# Autodesk Inventor assembly: 8163946 CMMT-ST-C8-1C-MP-S0---(high)
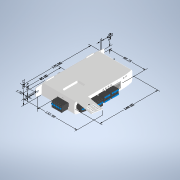
[picture p0: Inventor's stored thumbnail of the model, 180x180]
Saved by Autodesk Inventor 2021 (Build 250183000, 183)
## iProperties
Category: PARTsolutions
Company: FESTO
Created: 2026-04-23
Part Number: 8163946 CMMT-ST-C8-1C-MP-S0---(high)
Catalog Web Link: www.3dfindit.com
Description: CMMT-ST-servo drive
Vendor: FESTO
Document SubType Name: Assembly
Designer: psAdmin
Manufacturer: FESTO
Mass: 350 g
Surface Area: 725.969 cm^2
Volume: 348.658 cm^3
Density: 1.00385 g/cm^3
Title: 8163946 CMMT-ST-C8-1C-MP-S0
Author: Cadenas PARTsolutions
Comments: servo drive
PSOL_IDENT_0: {ATYP=ASSISTANT},{DATA=script=$CADENAS_DATA/23d-libs/festo/webfesto.vbb&M_FAMILY=CMMT&M_GROUP=01&M_P
PSOL_IDENT_1: ARTNO=8163946&IDCODE1=CMMT-ST-C8-1C-MP-S0&IDCODE2=&customer_number_cns=&MATES=1&LOD=HI&LOCKERP=0&SIN
PSOL_IDENT_2: GLEPART=1}
NB: 8163946 CMMT-ST-C8-1C-MP-S0---(high)
NN: CMMT-ST
NT: servo drive
NBSYN: $TNR. $TYP.---($LODLEVEL.)
LINA: 8163946 CMMT-ST-C8-1C-MP-S0
CATALOG: Festo
TNR: 8163946
TYP: CMMT-ST-C8-1C-MP-S0
LODLEVEL: High
CNSMASSEXACT: 0.35
GTIN: 4052568631956
SUPPLIER: FESTO
ARTICLENO: 8163946 CMMT-ST-C8-1C-MP-S0---(high)
BOMINFO: 8163946 CMMT-ST-C8-1C-MP-S0
CREATOR: CADENAS GmbH
## Documents named in this file (9)
- e:\temp\worker_COMMON_66\temp\tmp_7696_12_FVe9l\format_0\8163946 CMMT-ST-C8-1C-MP-S0---(high).iam
- e:\temp\worker_COMMON_66\temp\tmp_7696_12_FVe9l\format_0\8163946 CMMT-ST-C8-1C-MP-S0---(highh).ipt
- e:\temp\worker_COMMON_66\temp\tmp_7696_12_FVe9l\format_0\1360395 VAME-P11-MK.ipt
- e:\temp\worker_COMMON_66\temp\tmp_7696_12_FVe9l\format_0\DIN-912 - M4x5(F).ipt
- e:\temp\worker_COMMON_66\temp\tmp_7696_12_FVe9l\format_0\8079510 10GD-2RR3,5-CLP-CBL.ipt
- e:\temp\worker_COMMON_66\temp\tmp_7696_12_FVe9l\format_0\8079513 8GD-2RR3,5-CLP-CBL.ipt
- e:\temp\worker_COMMON_66\temp\tmp_7696_12_FVe9l\format_0\8079509 6GD-1RR5,08-CLP-CBL.ipt
- e:\temp\worker_COMMON_66\temp\tmp_7696_12_FVe9l\format_0\8079508 3GD-1RR3_5-CLP-CBL---(2).ipt
- e:\temp\worker_COMMON_66\temp\tmp_7696_12_FVe9l\format_0\8169608 5GD-1RR5,08-CLP-CBL.ipt
## Components (8 placed, 8 different names)
1. 8163946 CMMT-ST-C8-1C-MP-S0---(highh):1 — IP1_XY@1 <-> N_XY@2, IP1_Z@1 <-> N_Z@2, IP1_YZ@1 <-> N_YZ@2, P1_XY@1 <-> CP1_XY@4, P1_Z@1 <-> CP1_Z@4, P1_YZ@1 <-> CP1_YZ@4, P2_XY@1 <-> CP1_XY@5, P2_Z@1 <-> CP1_Z@5, P2_YZ@1 <-> CP1_YZ@5, P3_XY@1 <-> CP1_XY@6, P3_Z@1 <-> CP1_Z@6, P3_YZ@1 <-> CP1_YZ@6, P4_XY@1 <-> CP1_XY@7, P4_Z@1 <-> CP1_Z@7, P4_YZ@1 <-> CP1_YZ@7, P5_XY@1 <-> CP1_XY@8, P5_Z@1 <-> CP1_Z@8, P5_YZ@1 <-> CP1_YZ@8
2. 1360395 VAME-P11-MK:1 — IP1_XY@1 <-> N_XY@2, IP1_Z@1 <-> N_Z@2, IP1_YZ@1 <-> N_YZ@2, B_XY@2 <-> ANBAU_XY@3, B_Z@2 <-> ANBAU_Z@3, B_YZ@2 <-> ANBAU_YZ@3
3. DIN-912 - M4x5(F):1 — B_XY@2 <-> ANBAU_XY@3, B_Z@2 <-> ANBAU_Z@3, B_YZ@2 <-> ANBAU_YZ@3
4. 8079510 10GD-2RR3,5-CLP-CBL:1 — P1_XY@1 <-> CP1_XY@4, P1_Z@1 <-> CP1_Z@4, P1_YZ@1 <-> CP1_YZ@4
5. 8079513 8GD-2RR3,5-CLP-CBL:1 — P2_XY@1 <-> CP1_XY@5, P2_Z@1 <-> CP1_Z@5, P2_YZ@1 <-> CP1_YZ@5
6. 8079509 6GD-1RR5,08-CLP-CBL:1 — P3_XY@1 <-> CP1_XY@6, P3_Z@1 <-> CP1_Z@6, P3_YZ@1 <-> CP1_YZ@6
7. 8079508 3GD-1RR3_5-CLP-CBL---(2):1 — P4_XY@1 <-> CP1_XY@7, P4_Z@1 <-> CP1_Z@7, P4_YZ@1 <-> CP1_YZ@7
8. 8169608 5GD-1RR5,08-CLP-CBL:1 — P5_XY@1 <-> CP1_XY@8, P5_Z@1 <-> CP1_Z@8, P5_YZ@1 <-> CP1_YZ@8
## Relationships (21: Mate 13, Angle 7, Flush 1)
- IP1_XY@1 <-> N_XY@2 [Mate] (1.35 mm): 8163946 CMMT-ST-C8-1C-MP-S0---(highh):1 ↔ 1360395 VAME-P11-MK:1
- IP1_Z@1 <-> N_Z@2 [Mate]: 8163946 CMMT-ST-C8-1C-MP-S0---(highh):1 ↔ 1360395 VAME-P11-MK:1
- IP1_YZ@1 <-> N_YZ@2 [Angle] (0 deg): 8163946 CMMT-ST-C8-1C-MP-S0---(highh):1 ↔ 1360395 VAME-P11-MK:1
- B_XY@2 <-> ANBAU_XY@3 [Flush]: 1360395 VAME-P11-MK:1 ↔ DIN-912 - M4x5(F):1
- B_Z@2 <-> ANBAU_Z@3 [Mate]: 1360395 VAME-P11-MK:1 ↔ DIN-912 - M4x5(F):1
- B_YZ@2 <-> ANBAU_YZ@3 [Angle] (0 deg): 1360395 VAME-P11-MK:1 ↔ DIN-912 - M4x5(F):1
- P1_XY@1 <-> CP1_XY@4 [Mate]: 8163946 CMMT-ST-C8-1C-MP-S0---(highh):1 ↔ 8079510 10GD-2RR3,5-CLP-CBL:1
- P1_Z@1 <-> CP1_Z@4 [Mate]: 8163946 CMMT-ST-C8-1C-MP-S0---(highh):1 ↔ 8079510 10GD-2RR3,5-CLP-CBL:1
- P1_YZ@1 <-> CP1_YZ@4 [Angle] (0 deg): 8163946 CMMT-ST-C8-1C-MP-S0---(highh):1 ↔ 8079510 10GD-2RR3,5-CLP-CBL:1
- P2_XY@1 <-> CP1_XY@5 [Mate]: 8163946 CMMT-ST-C8-1C-MP-S0---(highh):1 ↔ 8079513 8GD-2RR3,5-CLP-CBL:1
- P2_Z@1 <-> CP1_Z@5 [Mate]: 8163946 CMMT-ST-C8-1C-MP-S0---(highh):1 ↔ 8079513 8GD-2RR3,5-CLP-CBL:1
- P2_YZ@1 <-> CP1_YZ@5 [Angle] (0 deg): 8163946 CMMT-ST-C8-1C-MP-S0---(highh):1 ↔ 8079513 8GD-2RR3,5-CLP-CBL:1
- P3_XY@1 <-> CP1_XY@6 [Mate]: 8163946 CMMT-ST-C8-1C-MP-S0---(highh):1 ↔ 8079509 6GD-1RR5,08-CLP-CBL:1
- P3_Z@1 <-> CP1_Z@6 [Mate]: 8163946 CMMT-ST-C8-1C-MP-S0---(highh):1 ↔ 8079509 6GD-1RR5,08-CLP-CBL:1
- P3_YZ@1 <-> CP1_YZ@6 [Angle] (0 deg): 8163946 CMMT-ST-C8-1C-MP-S0---(highh):1 ↔ 8079509 6GD-1RR5,08-CLP-CBL:1
- P4_XY@1 <-> CP1_XY@7 [Mate]: 8163946 CMMT-ST-C8-1C-MP-S0---(highh):1 ↔ 8079508 3GD-1RR3_5-CLP-CBL---(2):1
- P4_Z@1 <-> CP1_Z@7 [Mate]: 8163946 CMMT-ST-C8-1C-MP-S0---(highh):1 ↔ 8079508 3GD-1RR3_5-CLP-CBL---(2):1
- P4_YZ@1 <-> CP1_YZ@7 [Angle] (0 deg): 8163946 CMMT-ST-C8-1C-MP-S0---(highh):1 ↔ 8079508 3GD-1RR3_5-CLP-CBL---(2):1
- P5_XY@1 <-> CP1_XY@8 [Mate]: 8163946 CMMT-ST-C8-1C-MP-S0---(highh):1 ↔ 8169608 5GD-1RR5,08-CLP-CBL:1
- P5_Z@1 <-> CP1_Z@8 [Mate]: 8163946 CMMT-ST-C8-1C-MP-S0---(highh):1 ↔ 8169608 5GD-1RR5,08-CLP-CBL:1
- P5_YZ@1 <-> CP1_YZ@8 [Angle] (0 deg): 8163946 CMMT-ST-C8-1C-MP-S0---(highh):1 ↔ 8169608 5GD-1RR5,08-CLP-CBL:1
